# Autodesk Inventor assembly: motor_MIROR1
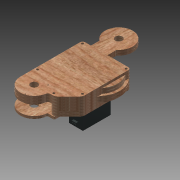
[picture p0: Inventor's stored thumbnail of the model, 180x180]
Saved by Autodesk Inventor 2015 (Build 190159000, 159)
## iProperties
Created: 2016-02-03
Part Number: motor_MIROR1
Document SubType Name: Assembly
Designer: david
Author: david
## Documents named in this file (11)
- Z:\gip\Inventor\generatie 7\motor v2\motor_MIROR1.iam
- Z:\gip\Inventor\generatie 7\motor v2\p1_MIROR1.ipt
- Z:\gip\Inventor\generatie 7\motor v2\p2_MIROR1.ipt
- Z:\gip\Inventor\generatie 7\motor v2\p3_MIROR1.ipt
- Z:\gip\Inventor\generatie 7\motor v2\p5_MIROR1.ipt
- Z:\gip\Inventor\generatie 7\motor v2\servo\block_MIROR1.ipt
- Z:\gip\Inventor\generatie 7\motor v2\servo\tang_MIROR1.ipt
- Z:\gip\Inventor\generatie 7\old\Motor\tanden2_MIROR1.ipt
- Z:\gip\Inventor\generatie 7\motor v2\tandwiel\tandwiel_MIROR1.iam
- Z:\gip\Inventor\generatie 7\motor v2\p5 big_MIROR.ipt
- Z:\gip\Inventor\generatie 7\motor v2\p6_MIROR1.ipt
## Components (13 placed, 10 different names)
1. p1_MIROR1:1 — Flush:2, Mate:1, Flush:16, Flush:4, Flush:18
2. p2_MIROR1:1 — Flush:2, Mate:1, Mate:22, Mate:2, Flush:5
3. p2_MIROR1:2 — Flush:16, Mate:22, Flush:4, Mate:2, Mate:23, Mate:3, Mate:15, Mate:21, Flush:20
4. p3_MIROR1:1 — Mate:23, Flush:5, Mate:3, Mate:13, Mate:33, Mate:32
5. p5_MIROR1:1 — Flush:18, Mate:31, Mate:30, Mate:29, Flush:25, Mate:42, Flush:26, Mate:40, Mate:39, Mate:38
6. block_MIROR1:1 — Mate:31, Mate:30, Mate:29, Mate:11, Mate:10
7. tang_MIROR1:1 — Mate:11, Mate:10, Mate:43, Mate:18
8. tanden2_MIROR1:1 — Mate:15, Mate:13, Rotation/Translation:1, Mate:20, Flush:13, Mate:19
9. tandwiel_MIROR1:1 [sub-assembly] — Mate:43, Mate:18, Rotation/Translation:1, Flush:19
10. tanden2_MIROR1:2 — Flush:19, Mate:21, Mate:20, Flush:13, Mate:19
11. p3_MIROR1:2 — Flush:25, Mate:33, Flush:20, Mate:32, Flush:24, Flush:23, Mate:41
12. p5 big_MIROR:1 — Mate:42, Flush:26, Flush:24, Flush:23, Mate:41
13. p6_MIROR1:1 — Mate:40, Mate:39, Mate:38
## Relationships (37: Mate 24, Flush 12, RelateRotateTranslate 1)
- Flush:2: p1_MIROR1:1 ↔ p2_MIROR1:1
- Mate:1: p1_MIROR1:1 ↔ p2_MIROR1:1
- Flush:16: p1_MIROR1:1 ↔ p2_MIROR1:2
- Mate:22: p2_MIROR1:1 ↔ p2_MIROR1:2
- Flush:4: p1_MIROR1:1 ↔ p2_MIROR1:2
- Mate:2: p2_MIROR1:1 ↔ p2_MIROR1:2
- Mate:23: p2_MIROR1:2 ↔ p3_MIROR1:1
- Flush:5: p2_MIROR1:1 ↔ p3_MIROR1:1
- Mate:3: p2_MIROR1:2 ↔ p3_MIROR1:1
- Flush:18: p1_MIROR1:1 ↔ p5_MIROR1:1
- Mate:31: p5_MIROR1:1 ↔ block_MIROR1:1
- Mate:30: p5_MIROR1:1 ↔ block_MIROR1:1
- Mate:29: p5_MIROR1:1 ↔ block_MIROR1:1
- Mate:11: block_MIROR1:1 ↔ tang_MIROR1:1
- Mate:10: block_MIROR1:1 ↔ tang_MIROR1:1
- Mate:15: p2_MIROR1:2 ↔ tanden2_MIROR1:1
- Mate:13: p3_MIROR1:1 ↔ tanden2_MIROR1:1
- Mate:43: tang_MIROR1:1 ↔ tandwiel_MIROR1:1
- Mate:18: tang_MIROR1:1 ↔ tandwiel_MIROR1:1
- Rotation/Translation:1 [RelateRotateTranslate] (100 mm): tanden2_MIROR1:1 ↔ tandwiel_MIROR1:1
- Flush:19: tandwiel_MIROR1:1 ↔ tanden2_MIROR1:2
- Mate:21: p2_MIROR1:2 ↔ tanden2_MIROR1:2
- Mate:20: tanden2_MIROR1:1 ↔ tanden2_MIROR1:2
- Flush:13: tanden2_MIROR1:1 ↔ tanden2_MIROR1:2
- Mate:19: tanden2_MIROR1:1 ↔ tanden2_MIROR1:2
- Flush:25: p5_MIROR1:1 ↔ p3_MIROR1:2
- Mate:33: p3_MIROR1:1 ↔ p3_MIROR1:2
- Flush:20: p2_MIROR1:2 ↔ p3_MIROR1:2
- Mate:32: p3_MIROR1:1 ↔ p3_MIROR1:2
- Mate:42: p5_MIROR1:1 ↔ p5 big_MIROR:1
- Flush:26: p5_MIROR1:1 ↔ p5 big_MIROR:1
- Flush:24: p3_MIROR1:2 ↔ p5 big_MIROR:1
- Flush:23: p3_MIROR1:2 ↔ p5 big_MIROR:1
- Mate:41: p3_MIROR1:2 ↔ p5 big_MIROR:1
- Mate:40: p5_MIROR1:1 ↔ p6_MIROR1:1
- Mate:39: p5_MIROR1:1 ↔ p6_MIROR1:1
- Mate:38: p5_MIROR1:1 ↔ p6_MIROR1:1
